# Autodesk Inventor assembly: carriage
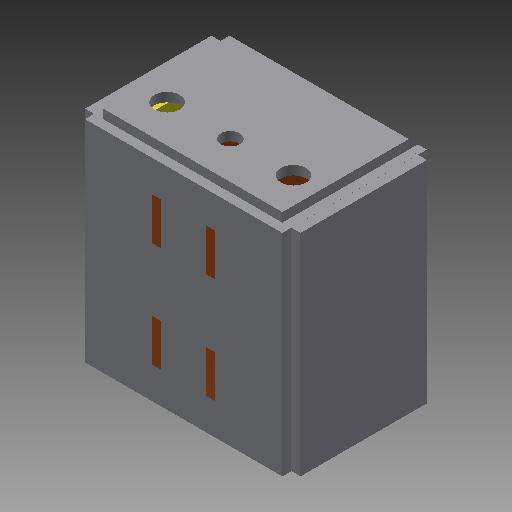
[picture p0: Inventor's stored thumbnail of the model, 512x512]
Saved by Autodesk Inventor 2017 (Build 210142000, 142)
## iProperties
Created: 2015-10-11
Part Number: carriage
Document SubType Name: Assembly
Designer: daniel
Author: daniel
## Documents named in this file (4)
- C:\Users\daniel\Documents\GitHub\cardboard-stage-metric\stage\carriage.iam
- C:\Users\daniel\Documents\GitHub\cardboard-stage-metric\stage\c1.iam
- C:\Users\daniel\Documents\GitHub\cardboard-stage-metric\stage\c2.iam
- C:\Users\daniel\Documents\GitHub\cardboard-stage-metric\stage\carriage_internal.iam
## Components (3 placed, 3 different names)
1. c1:1 [sub-assembly] — Flush:1, Mate:2, Mate:3
2. c2:1 [sub-assembly] — Mate:5, Mate:6, Mate:7
3. carriage_internal:1 [sub-assembly] — Flush:1, Mate:2, Mate:3, Mate:5, Mate:6, Mate:7
## Relationships (6: Mate 5, Flush 1)
- Flush:1: c1:1 ↔ carriage_internal:1
- Mate:2: c1:1 ↔ carriage_internal:1
- Mate:3: c1:1 ↔ carriage_internal:1
- Mate:5: c2:1 ↔ carriage_internal:1
- Mate:6: c2:1 ↔ carriage_internal:1
- Mate:7: c2:1 ↔ carriage_internal:1
